# Autodesk Inventor assembly: All
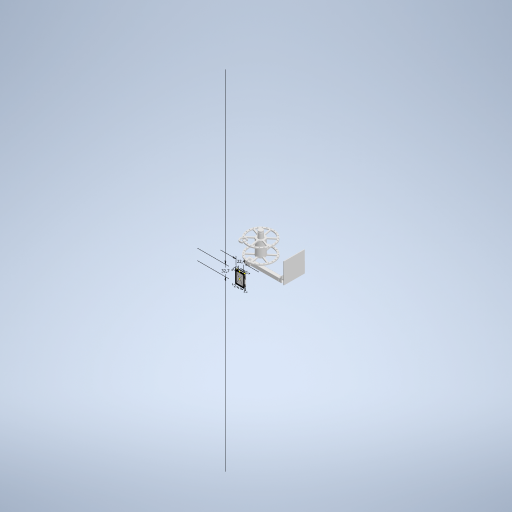
[picture p0: Inventor's stored thumbnail of the model, 512x512]
Saved by Autodesk Inventor 2024 (Build 280153000, 153)
## iProperties
Created: 2024-01-02
Part Number: All
Document SubType Name: Assembly
Designer: chris
Author: chris
## Documents named in this file (7)
- C:\Users\chris\OneDrive\alles andere\Dokumente\Inventor\CardWheel\All.iam
- C:\Users\chris\OneDrive\alles andere\Dokumente\Inventor\CardWheel\Wheel\WheelV1.ipt
- C:\Users\chris\OneDrive\alles andere\Dokumente\Inventor\CardWheel\Stand\Stand\StandV11.ipt
- C:\Users\chris\OneDrive\alles andere\Dokumente\Inventor\CardWheel\C-Clip\C-ClipV1.ipt
- C:\Users\chris\OneDrive\alles andere\Dokumente\Inventor\SwitchCardHolder\SwitchCardHolderNoHoldersSupportsInventor055.ipt
- C:\Users\chris\OneDrive\alles andere\Dokumente\Inventor\CardWheel\Stand\Ground\GroundV11.ipt
- C:\Users\chris\OneDrive\alles andere\Dokumente\Inventor\CardWheel\Stand\Axis\AxisV3.ipt
## Components (6 placed, 6 different names)
1. WheelV1:1 — Passend:1, Fluchtend:1
2. StandV11:1
3. C-ClipV1:1
4. SwitchCardHolderNoHoldersSupportsInventor055:1
5. GroundV11:1
6. AxisV3:1 — Passend:1, Fluchtend:1
## Relationships (2: Mate 1, Flush 1)
- Passend:1 [Mate]: WheelV1:1 ↔ AxisV3:1
- Fluchtend:1 [Flush] (-20 mm): WheelV1:1 ↔ AxisV3:1
